# Autodesk Inventor assembly: Lift
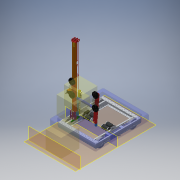
[picture p0: Inventor's stored thumbnail of the model, 180x180]
Saved by Autodesk Inventor 2017 SP1 (Build 210196100, 196)
## iProperties
Created: 2018-01-18
Part Number: Lift
Document SubType Name: Assembly
Designer: Ben
Mass: 3205.42 g
Surface Area: 51290.7 cm^2
Volume: 100604 cm^3
Density: 0.0318616 g/cm^3
Author: Ben
## Documents named in this file (21)
- C:\Users\Ben\Desktop\Projects\2018 Robot\Cube Lift\Lift 2.iam
- C:\Users\Ben\Desktop\Projects\2018 Robot\Cube Lift\Rail.ipt
- C:\Users\Ben\Desktop\Projects\2018 Robot\Chassis\2018_chassis.iam
- C:\Users\Ben\Desktop\Projects\2018 Robot\Cube Lift\roller bushing.iam
- C:\Users\Ben\Desktop\Projects\2018 Robot\Cube Lift\cube.ipt
- C:\Users\Ben\Desktop\Projects\2018 Robot\Cube Lift\carriage plate square 2.ipt
- C:\Users\Ben\Desktop\Projects\2018 Robot\Cube Lift\support plate 2.ipt
- C:\Users\Ben\Desktop\Projects\2018 Robot\Cube Lift\top pully bracket.ipt
- C:\Users\Ben\Desktop\Projects\2018 Robot\Cube Lift\pulley XL 1in.ipt
- C:\Users\Ben\Desktop\Projects\2018 Robot\Cube Lift\pulley XL 1.375in 2.ipt
- C:\Users\Ben\Desktop\Projects\2018 Robot\Cube Lift\first stage belt.ipt
- C:\Users\Ben\Desktop\Projects\2018 Robot\Cube Lift\upper anchor.ipt
- C:\Users\Ben\Desktop\Projects\2018 Robot\Cube Lift\top pully bracket 2.ipt
- C:\Users\Ben\Desktop\Projects\2018 Robot\Cube Lift\second stage belt 2.ipt
- C:\Users\Ben\Desktop\Projects\2018 Robot\Cube Lift\carriage plate for intake.ipt
- C:\Users\Ben\Desktop\Projects\2018 Robot\Cube Intake\Intake.iam
- C:\Users\Ben\Desktop\Projects\2018 Robot\Cube Lift\cylinder arm.ipt
- C:\Users\Ben\Desktop\Projects\2018 Robot\Cube Lift\cylinder body.ipt
- C:\Users\Ben\Desktop\Projects\2018 Robot\Cube Lift\cylinder piston.ipt
- C:\Users\Ben\Desktop\Projects\2018 Robot\Cube Lift\line pulley.ipt
- C:\Users\Ben\Desktop\Projects\2018 Robot\Cube Lift\outside carriage plate.ipt
## Components (28 placed, 20 different names)
1. Rail:1 — Mate:13, Flush:15, Flush:16, Mate:20, Mate:21, Mate:22, Mate:23, Mate:30, Flush:26, Flush:27, Flush:28, Flush:29, Mate:39, Flush:30, Angle:2, Flush:33, Mate:44, Flush:43, Mate:72
2. 2018_chassis:1 [sub-assembly] — Mate:1, Flush:3, Flush:4, Mate:13, Flush:15, Flush:21, Flush:46, Mate:64, Flush:49
3. Rail:3 — Mate:5, Flush:16, Mate:24, Flush:34, Mate:48, Flush:35, Angle:4, Mate:50, Flush:40, Flush:41, Flush:42, Mate:54, Mate:55
4. roller bushing:1 [sub-assembly] — Mate:38, Flush:28
5. cube:1 — Flush:5
6. carriage plate square 2:1 — Mate:5, Mate:20, Mate:21, Mate:22, Mate:23, Mate:24, Mate:36, Mate:37, Mate:38, Mate:66, Mate:67, Mate:73, Mate:74
7. roller bushing:2 [sub-assembly] — Mate:36, Flush:26
8. roller bushing:3 [sub-assembly] — Mate:37, Flush:27
9. roller bushing:4 [sub-assembly] — Flush:42, Insert:11
10. roller bushing:5 [sub-assembly] — Mate:53, Flush:40
11. roller bushing:6 [sub-assembly] — Flush:41, Mate:56
12. support plate 2:1 — Mate:30, Insert:8, Flush:43, Mate:64
13. top pully bracket:1 — Flush:29, Mate:39, Flush:30, Mate:40, Flush:31, Mate:65
14. pulley XL 1in:1 — Insert:8, Insert:9
15. pulley XL 1.375in 2:1 — Mate:40, Flush:31
16. first stage belt:1 — Insert:9, Angle:2
17. upper anchor:1 — Flush:33, Mate:44, Mate:65
18. top pully bracket 2:1 — Flush:34, Mate:48, Flush:35, Mate:70, Mate:71
19. second stage belt 2:1 — Angle:4, Mate:68, Mate:69
20. carriage plate for intake:1 — Mate:50, Mate:53, Mate:54, Mate:55, Insert:11, Mate:56, Mate:57, Insert:12, Insert:16, Flush:49
21. Intake:1 [sub-assembly] — Flush:45, Mate:57, Insert:15
22. cylinder arm:1 — Insert:12, Mate:62, Insert:16
23. cube:2 — Mate:58, Flush:48
24. cylinder body:1 — Mate:62, Mate:63
25. cylinder piston:1 — Mate:63, Insert:15
26. line pulley:1 — Mate:66, Mate:67, Mate:68, Mate:69
27. line pulley:2 — Mate:70, Mate:71
28. outside carriage plate:1 — Mate:72, Mate:73, Mate:74
## Relationships (70: Mate 36, Flush 26, Insert 6, Angle 2)
- Mate:1 (44.45 mm): 2018_chassis:1
- Flush:3: 2018_chassis:1
- Flush:4: 2018_chassis:1
- Flush:5: cube:1
- Mate:5: Rail:3 ↔ carriage plate square 2:1
- Mate:13: Rail:1 ↔ 2018_chassis:1
- Flush:15 (177.8 mm): Rail:1 ↔ 2018_chassis:1
- Flush:16: Rail:1 ↔ Rail:3
- Mate:20 (9.525 mm): Rail:1 ↔ carriage plate square 2:1
- Mate:21 (13.9192 mm): Rail:1 ↔ carriage plate square 2:1
- Mate:22 (13.9192 mm): Rail:1 ↔ carriage plate square 2:1
- Mate:23 (13.9192 mm): Rail:1 ↔ carriage plate square 2:1
- Mate:24: Rail:3 ↔ carriage plate square 2:1
- Flush:18 (1397 mm)
- Flush:19 (1930.4 mm)
- Flush:20 (2184.4 mm)
- Flush:21 (-558.8 mm): 2018_chassis:1
- Mate:30: Rail:1 ↔ support plate 2:1
- Mate:36: carriage plate square 2:1 ↔ roller bushing:2
- Flush:26 (-2.3622 mm): Rail:1 ↔ roller bushing:2
- Mate:37: carriage plate square 2:1 ↔ roller bushing:3
- Flush:27 (-2.3622 mm): Rail:1 ↔ roller bushing:3
- Mate:38: roller bushing:1 ↔ carriage plate square 2:1
- Flush:28 (2.3622 mm): Rail:1 ↔ roller bushing:1
- Flush:29 (-1.5875 mm): Rail:1 ↔ top pully bracket:1
- Mate:39: Rail:1 ↔ top pully bracket:1
- Flush:30 (6.35 mm): Rail:1 ↔ top pully bracket:1
- Insert:8 (4.7625 mm): support plate 2:1 ↔ pulley XL 1in:1
- Mate:40: top pully bracket:1 ↔ pulley XL 1.375in 2:1
- Flush:31: top pully bracket:1 ↔ pulley XL 1.375in 2:1
- Insert:9 (1.5875 mm): pulley XL 1in:1 ↔ first stage belt:1
- Angle:2 (0 deg): Rail:1 ↔ first stage belt:1
- Flush:33: Rail:1 ↔ upper anchor:1
- Mate:44: Rail:1 ↔ upper anchor:1
- Flush:34 (-1.5875 mm): Rail:3 ↔ top pully bracket 2:1
- Mate:48: Rail:3 ↔ top pully bracket 2:1
- Flush:35 (-6.35 mm): Rail:3 ↔ top pully bracket 2:1
- Angle:4 (0 deg): Rail:3 ↔ second stage belt 2:1
- Mate:50 (2.3622 mm): Rail:3 ↔ carriage plate for intake:1
- Mate:53: roller bushing:5 ↔ carriage plate for intake:1
- Flush:40 (-2.3622 mm): Rail:3 ↔ roller bushing:5
- Flush:41 (-2.3622 mm): Rail:3 ↔ roller bushing:6
- Flush:42 (-2.3622 mm): Rail:3 ↔ roller bushing:4
- Mate:54 (13.9192 mm): Rail:3 ↔ carriage plate for intake:1
- Mate:55 (13.9192 mm): Rail:3 ↔ carriage plate for intake:1
- Insert:11: roller bushing:4 ↔ carriage plate for intake:1
- Mate:56: roller bushing:6 ↔ carriage plate for intake:1
- Flush:43: Rail:1 ↔ support plate 2:1
- Flush:45: Intake:1
- Flush:46 (406.4 mm): 2018_chassis:1
- Mate:57: carriage plate for intake:1 ↔ Intake:1
- Insert:12: carriage plate for intake:1 ↔ cylinder arm:1
- Mate:58: cube:2
- Flush:48: cube:2
- Mate:62: cylinder arm:1 ↔ cylinder body:1
- Mate:63: cylinder body:1 ↔ cylinder piston:1
- Insert:15 (1.5875 mm): Intake:1 ↔ cylinder piston:1
- Mate:64 (-11.6078 mm): 2018_chassis:1 ↔ support plate 2:1
- Insert:16: carriage plate for intake:1 ↔ cylinder arm:1
- Flush:49 (-158.75 mm): 2018_chassis:1 ↔ carriage plate for intake:1
- Mate:65: top pully bracket:1 ↔ upper anchor:1
- Mate:66: carriage plate square 2:1 ↔ line pulley:1
- Mate:67 (3.175 mm): carriage plate square 2:1 ↔ line pulley:1
- Mate:68: second stage belt 2:1 ↔ line pulley:1
- Mate:69 (0.7937 mm): second stage belt 2:1 ↔ line pulley:1
- Mate:70: top pully bracket 2:1 ↔ line pulley:2
- Mate:71 (4.7625 mm): top pully bracket 2:1 ↔ line pulley:2
- Mate:72 (2.3622 mm): Rail:1 ↔ outside carriage plate:1
- Mate:73: carriage plate square 2:1 ↔ outside carriage plate:1
- Mate:74: carriage plate square 2:1 ↔ outside carriage plate:1
